# Autodesk Inventor assembly: Scale Platform
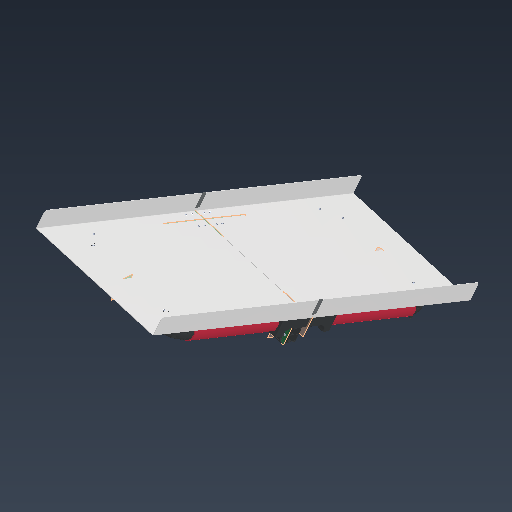
[picture p0: Inventor's stored thumbnail of the model, 512x512]
Saved by Autodesk Inventor 2021 (Build 250183000, 183)
## iProperties
Created: 2021-07-21
Part Number: Scale Platform
Document SubType Name: Assembly
Designer: max
Author: max
## Documents named in this file (18)
- C:\Users\max\Desktop\Vex\TiP FieldCAD\Scales\Scale Platform.iam
- C:\Users\max\Desktop\Vex\Vex 21-22\Field CAD\276-7048-104 Rev6.ipt
- C:\Users\max\Desktop\Vex\TiP FieldCAD\Scales\Scale Platform Corner Pipe Coupler.ipt
- C:\Users\max\Desktop\Vex\TiP FieldCAD\Scales\Scale Platform Poly.ipt
- C:\Users\max\Desktop\Vex\TiP FieldCAD\Scales\Scale Pipe Short Red.ipt
- C:\Users\max\Desktop\Vex\TiP FieldCAD\Scales\Scale Pipe Long Red.ipt
- C:\Users\max\Desktop\Vex\Library 1.2\Structure\Standoff\Standoff 2.ipt
- C:\Users\max\Desktop\Vex\Library 1.2\Structure\Standoff.ipt
- C:\Users\max\Desktop\Vex\Library 1.2\Structure\Hardware\Screw Steel - Star\Screw 8-32 Steel .500.ipt
- C:\Users\max\Desktop\Vex\Library 1.2\Structure\Hardware\Screw Steel - Star.ipt
- C:\Users\max\Desktop\Vex\Library 1.2\Structure\Hardware\Screw Steel - Star\Screw 8-32 Steel 1.500.ipt
- C:\Users\max\Desktop\Vex\Library 1.2\Structure\Hardware\Nut Nylock.ipt
- C:\Users\max\Desktop\Vex\Library 1.2\Structure\Standoff\Standoff .75.ipt
- C:\Users\max\Desktop\Vex\TiP FieldCAD\Scales\Scale Center Beam.ipt
- C:\Users\max\Desktop\Vex\TiP FieldCAD\Scales\Scale Pivot Coupler.ipt
- C:\Users\max\Desktop\Vex\Library 1.2\Structure\Standoff\Standoff 1.5.ipt
- C:\Users\max\Desktop\Vex\Library 1.2\Structure\Hardware\Screw Steel - Star\Screw 8-32 Steel .375.ipt
- C:\Users\max\Desktop\Vex\TiP FieldCAD\Scales\Scale Platform Poly Clip.ipt
## Components (85 placed, 16 different names)
1. 276-7048-104 Rev6_451
2. Scale Platform Corner Pipe Coupler:1
3. Scale Platform Poly:1
4. Scale Pipe Short Red:1
5. Scale Pipe Long Red:1
6. Scale Platform Corner Pipe Coupler:2
7. 276-7048-104 Rev6:2
8. Scale Pipe Long Red:2
9. Standoff 2:1
10. Screw 8-32 Steel .500:1
11. Screw 8-32 Steel .500:2
12. Standoff 2:2
13. Screw 8-32 Steel .500:3
14. Screw 8-32 Steel .500:4
15. Standoff 2:3
16. Screw 8-32 Steel .500:5
17. Screw 8-32 Steel .500:6
18. Standoff 2:4
19. Screw 8-32 Steel .500:7
20. Screw 8-32 Steel .500:8
21. Scale Platform Corner Pipe Coupler:3
22. Scale Pipe Short Red:2
23. Scale Pipe Long Red:3
24. Scale Platform Corner Pipe Coupler:4
25. Scale Pipe Long Red:4
26. Standoff 2:5
27. Screw 8-32 Steel .500:9
28. Screw 8-32 Steel .500:10
29. Standoff 2:6
30. Screw 8-32 Steel .500:11
31. Screw 8-32 Steel .500:12
32. Standoff 2:7
33. Screw 8-32 Steel .500:13
34. Screw 8-32 Steel .500:14
35. Standoff 2:8
36. Screw 8-32 Steel .500:15
37. Screw 8-32 Steel .500:16
38. Screw 8-32 Steel 1.500:17
39. Nut Nylock:1
40. Screw 8-32 Steel 1.500:18
41. Nut Nylock:2
42. Screw 8-32 Steel 1.500:19
43. Nut Nylock:3
44. Screw 8-32 Steel 1.500:20
45. Nut Nylock:4
46. Screw 8-32 Steel 1.500:21
47. Nut Nylock:5
48. Screw 8-32 Steel 1.500:22
49. Nut Nylock:6
50. Screw 8-32 Steel 1.500:23
51. Nut Nylock:7
52. Screw 8-32 Steel 1.500:24
53. Nut Nylock:8
54. Scale Platform Poly:2
55. Screw 8-32 Steel 1.500:25
56. Nut Nylock:9
57. Screw 8-32 Steel 1.500:26
58. Nut Nylock:10
59. Screw 8-32 Steel 1.500:27
60. Nut Nylock:11
61. Screw 8-32 Steel 1.500:28
62. Nut Nylock:12
63. Screw 8-32 Steel 1.500:29
64. Nut Nylock:13
65. Screw 8-32 Steel 1.500:30
66. Nut Nylock:14
67. Screw 8-32 Steel 1.500:31
68. Nut Nylock:15
69. Screw 8-32 Steel 1.500:32
70. Nut Nylock:16
71. Standoff .75:9
72. Standoff .75:10
73. Standoff .75:11
74. Standoff .75:12
75. Scale Center Beam:1
76. Scale Pivot Coupler:1
77. Standoff 1.5:13
78. Screw 8-32 Steel .375:33
79. Screw 8-32 Steel .375:34
80. Scale Pivot Coupler:2
81. Standoff 1.5:14
82. Screw 8-32 Steel .375:35
83. Screw 8-32 Steel .375:36
84. Scale Platform Poly Clip:1
85. Scale Platform Poly Clip:2
## Relationships (67: Mate 50, Insert 8, Flush 7, Angle 2)
- [Angle] (0 deg): 276-7048-104 Rev6_451 ↔ Scale Platform Corner Pipe Coupler:1
- [Mate]: 276-7048-104 Rev6_451 ↔ Scale Pipe Long Red:1
- [Mate]: Scale Platform Corner Pipe Coupler:1 ↔ Scale Pipe Long Red:1
- [Mate]: Scale Platform Corner Pipe Coupler:1 ↔ Scale Pipe Long Red:1
- [Mate]: 276-7048-104 Rev6_451 ↔ Scale Pipe Long Red:1
- [Mate]: Scale Platform Corner Pipe Coupler:1 ↔ Scale Pipe Short Red:1
- [Mate]: Scale Platform Corner Pipe Coupler:1 ↔ Scale Pipe Short Red:1
- [Mate]: Scale Pipe Short Red:1 ↔ Scale Platform Corner Pipe Coupler:2
- [Mate]: Scale Pipe Short Red:1 ↔ Scale Platform Corner Pipe Coupler:2
- [Flush]: Scale Platform Corner Pipe Coupler:1 ↔ Scale Platform Corner Pipe Coupler:2
- [Mate]: Scale Platform Corner Pipe Coupler:2 ↔ Scale Pipe Long Red:2
- [Mate]: Scale Platform Corner Pipe Coupler:2 ↔ Scale Pipe Long Red:2
- [Mate]: 276-7048-104 Rev6:2 ↔ Scale Pipe Long Red:2
- [Mate]: 276-7048-104 Rev6:2 ↔ Scale Pipe Long Red:2
- [Flush]: 276-7048-104 Rev6_451 ↔ 276-7048-104 Rev6:2
- [Mate]: Standoff 2:1 ↔ Screw 8-32 Steel .500:1
- [Mate] (1.975 mm): Standoff 2:1 ↔ Screw 8-32 Steel .500:1
- [Mate]: Scale Platform Corner Pipe Coupler:1 ↔ Standoff 2:1
- [Mate]: Scale Platform Corner Pipe Coupler:1 ↔ Standoff 2:1
- [Mate]: Standoff 2:1 ↔ Screw 8-32 Steel .500:2
- [Mate] (1.975 mm): Standoff 2:1 ↔ Screw 8-32 Steel .500:2
- [Mate]: Standoff 2:2 ↔ Screw 8-32 Steel .500:3
- [Mate] (1.975 mm): Standoff 2:2 ↔ Screw 8-32 Steel .500:3
- [Mate]: Standoff 2:2 ↔ Screw 8-32 Steel .500:4
- [Mate] (1.975 mm): Standoff 2:2 ↔ Screw 8-32 Steel .500:4
- [Flush]: Scale Platform Corner Pipe Coupler:1 ↔ Standoff 2:1
- [Mate]: Scale Platform Corner Pipe Coupler:1 ↔ Standoff 2:2
- [Mate]: Scale Platform Corner Pipe Coupler:1 ↔ Standoff 2:2
- [Flush]: Scale Platform Corner Pipe Coupler:1 ↔ Standoff 2:2
- [Mate] (1.975 mm): Standoff 2:3 ↔ Screw 8-32 Steel .500:5
- [Mate]: Standoff 2:3 ↔ Screw 8-32 Steel .500:5
- [Mate] (1.975 mm): Standoff 2:3 ↔ Screw 8-32 Steel .500:6
- [Mate]: Standoff 2:3 ↔ Screw 8-32 Steel .500:6
- [Mate] (1.975 mm): Standoff 2:4 ↔ Screw 8-32 Steel .500:7
- [Mate]: Standoff 2:4 ↔ Screw 8-32 Steel .500:7
- [Mate] (1.975 mm): Standoff 2:4 ↔ Screw 8-32 Steel .500:8
- [Mate]: Standoff 2:4 ↔ Screw 8-32 Steel .500:8
- [Mate]: Screw 8-32 Steel 1.500:17 ↔ Nut Nylock:1
- [Mate] (25.9 mm): Screw 8-32 Steel 1.500:17 ↔ Nut Nylock:1
- [Insert]: Scale Platform Poly:1 ↔ 276-7048-104 Rev6:2
- [Mate]: Scale Platform Poly:1 ↔ 276-7048-104 Rev6:2
- [Insert]: Scale Platform Poly:1 ↔ Screw 8-32 Steel 1.500:17
- [Mate]: Screw 8-32 Steel 1.500:18 ↔ Nut Nylock:2
- [Mate] (25.9 mm): Screw 8-32 Steel 1.500:18 ↔ Nut Nylock:2
- [Mate]: Screw 8-32 Steel 1.500:19 ↔ Nut Nylock:3
- [Mate] (25.9 mm): Screw 8-32 Steel 1.500:19 ↔ Nut Nylock:3
- [Mate]: Screw 8-32 Steel 1.500:20 ↔ Nut Nylock:4
- [Mate] (25.9 mm): Screw 8-32 Steel 1.500:20 ↔ Nut Nylock:4
- [Insert]: Scale Platform Poly:1 ↔ Screw 8-32 Steel 1.500:18
- [Insert]: Scale Platform Poly:1 ↔ Screw 8-32 Steel 1.500:19
- [Insert]: Scale Platform Poly:1 ↔ Screw 8-32 Steel 1.500:20
- [Mate]: 276-7048-104 Rev6:2 ↔ Standoff .75:9
- [Mate]: 276-7048-104 Rev6:2 ↔ Standoff .75:10
- [Flush]: Standoff .75:9 ↔ Standoff .75:10
- [Mate]: 276-7048-104 Rev6:2 ↔ Standoff .75:10
- [Insert]: 276-7048-104 Rev6:2 ↔ Scale Center Beam:1
- [Mate]: 276-7048-104 Rev6:2 ↔ Scale Center Beam:1
- [Mate]: Scale Pivot Coupler:1 ↔ Standoff 1.5:13
- [Mate]: Scale Pivot Coupler:1 ↔ Standoff 1.5:13
- [Insert]: Scale Pivot Coupler:1 ↔ Screw 8-32 Steel .375:33
- [Insert]: Scale Pivot Coupler:1 ↔ Screw 8-32 Steel .375:34
- [Mate]: 276-7048-104 Rev6_451 ↔ Scale Pivot Coupler:1
- [Angle] (0 deg): 276-7048-104 Rev6_451 ↔ Scale Pivot Coupler:1
- [Flush]: 276-7048-104 Rev6_451 ↔ Scale Pivot Coupler:1
- [Mate] (0.127 mm): Scale Platform Poly:1 ↔ Scale Platform Poly Clip:1
- [Flush]: Scale Platform Poly:1 ↔ Scale Platform Poly Clip:1
- [Mate]: Scale Platform Poly:1 ↔ Scale Platform Poly Clip:1
## Named parameters: d107_d16 = 0 mm, d108_d15 = 0 mm, d109_d11 = 0 mm, d110_d12 = 0 mm, d18_d61 = 0 mm, d19_d62 = 1.975 mm, d71_d61 = 0 mm, d72_d62 = 1.975 mm, d73_d69 = 0 mm, d74_d70 = 1.975 mm, d92_d87 = 0 mm, d93_d88 = 25.9 mm, d94_d87 = 0 mm, d95_d88 = 25.9 mm, d96_d87 = 0 mm, d97_d88 = 25.9 mm
